# Autodesk Inventor assembly: prueba1
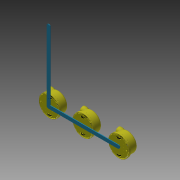
[picture p0: Inventor's stored thumbnail of the model, 180x180]
Saved by Autodesk Inventor 2015 (Build 190159000, 159)
## iProperties
Created: 2015-06-07
Part Number: prueba1
Document SubType Name: Assembly
Designer: david_000
Author: david_000
## Documents named in this file (3)
- C:\Users\david_000\Desktop\minibot-code\mechanics\prueba1.iam
- C:\Users\david_000\Desktop\minibot-code\mechanics\suelo_pruebas.ipt
- C:\Users\david_000\Desktop\minibot-code\mechanics\minibot.iam
## Components (4 placed, 2 different names)
1. suelo_pruebas:1 — Coincidencia:1, Coincidencia:2, Coincidencia:3
2. minibot:1 [sub-assembly] — Coincidencia:1, Coincidencia:2, Nivelación:1, Nivelación:4
3. minibot:2 [sub-assembly] — Nivelación:1, Nivelación:2, Nivelación:3, Nivelación:4
4. minibot:3 [sub-assembly] — Nivelación:2, Coincidencia:3, Nivelación:3
## Relationships (7: Flush 4, Mate 3)
- Coincidencia:1 [Mate]: suelo_pruebas:1 ↔ minibot:1
- Coincidencia:2 [Mate]: suelo_pruebas:1 ↔ minibot:1
- Nivelación:1 [Flush]: minibot:1 ↔ minibot:2
- Nivelación:2 [Flush]: minibot:2 ↔ minibot:3
- Coincidencia:3 [Mate]: suelo_pruebas:1 ↔ minibot:3
- Nivelación:3 [Flush]: minibot:2 ↔ minibot:3
- Nivelación:4 [Flush]: minibot:1 ↔ minibot:2
